# Autodesk Inventor assembly: Antenna assy
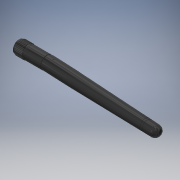
[picture p0: Inventor's stored thumbnail of the model, 180x180]
Saved by Autodesk Inventor 2019 (Build 230136000, 136)
## iProperties
Created: 2019-01-17
Part Number: Antenna assy
Document SubType Name: Assembly
Designer: Pulag
Author: Pulag
Sending System: SolidWorks 2016
Last Author: Condor
Last Saved: 2019-01-18
## Documents named in this file (3)
- C:\Users\Pulag\Documents\GitHub\24th_TDK_Project_D5\CAD\CAD file\nrf24l01p-pa-lna-1.snapshot.2\NRF24L01L + Antenna 2.4 GHz\Antenna assy.iam
- C:\Users\Pulag\Documents\GitHub\24th_TDK_Project_D5\CAD\CAD file\nrf24l01p-pa-lna-1.snapshot.2\NRF24L01L + Antenna 2.4 GHz\Antenna base.ipt
- C:\Users\Pulag\Documents\GitHub\24th_TDK_Project_D5\CAD\CAD file\nrf24l01p-pa-lna-1.snapshot.2\NRF24L01L + Antenna 2.4 GHz\Antenna top.ipt
## Components (2 placed, 2 different names)
1. Antenna base:1 — Mate:1, Mate:2
2. Antenna top:1 — Mate:1, Mate:2
## Relationships (2: Mate 2)
- Mate:1: Antenna base:1 ↔ Antenna top:1
- Mate:2: Antenna base:1 ↔ Antenna top:1
